# Autodesk Inventor assembly: папус для вари
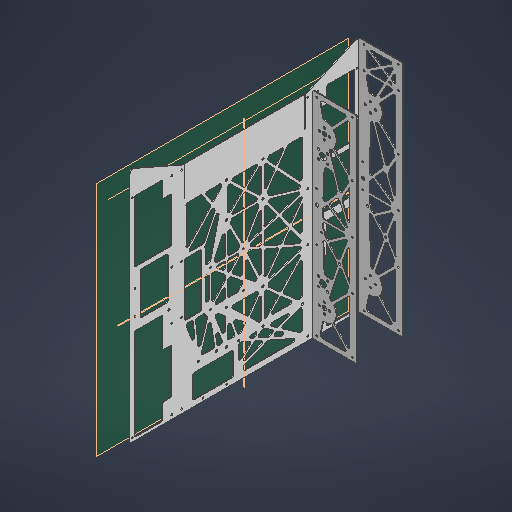
[picture p0: Inventor's stored thumbnail of the model, 512x512]
Saved by Autodesk Inventor 2026.2 (Build 302298000, 298)
## iProperties
Created: 2025-11-01
Part Number: папус для вари
Document SubType Name: Assembly
Designer: Phantom
Author: Phantom
## Documents named in this file (32)
- C:\Users\Phantom\Desktop\Phantom16950\папус для вари.iam
- C:\Users\Phantom\Desktop\Phantom16950\дно 25-26.ipt
- C:\Users\Phantom\Desktop\Phantom16950\кб 2025-2026.ipt
- C:\Users\Phantom\Desktop\Phantom16950\угол 25-26.ipt
- C:\Users\Phantom\Desktop\Phantom16950\кб 2025-2026 2 часть.ipt
- C:\Users\Phantom\Desktop\Phantom16950\кб 2025-2026 2 часть_MIR.ipt
- C:\Users\Phantom\Desktop\Phantom16950\ВЕРХ 25-26.ipt
- C:\Users\Phantom\Desktop\Phantom16950\наклон.ipt
- C:\Users\Phantom\Desktop\Phantom16950\цепь_MIR4.iam
- C:\Users\Phantom\Desktop\Phantom16950\КОЛЕСО_MIR_MIR3.ipt
- C:\Users\Phantom\Desktop\Phantom16950\арина треугольник 2.ipt
- C:\Users\Phantom\Desktop\Phantom16950\5203-2402-0014 assembly\5203-2402-0014 assembly.iam
- C:\Users\Phantom\Desktop\Phantom16950\шестерня шеврон кб 25-26.ipt
- C:\Users\Phantom\Desktop\Phantom16950\шестерня ответная 2.0 кб 25-26\шестерня ответная 2.0 кб 25-26.ipt
- C:\Users\Phantom\Desktop\Phantom16950\цепь_MIR4_MIR.iam
- C:\Users\Phantom\Desktop\Phantom16950\КОЛЕСО_MIR_MIR3_MIR.ipt
- C:\Users\Phantom\Desktop\Phantom16950\шестерня шеврон кб 25-26_MIR.ipt
- C:\Users\Phantom\Desktop\Phantom16950\шестерня ответная 2.0 кб 25-26\шестерня ответная 2.0 кб 25-26_MIR.ipt
- C:\Users\Phantom\Desktop\Phantom16950\цепь_MIR4_MIR1.iam
- C:\Users\Phantom\Desktop\Phantom16950\КОЛЕСО_MIR_MIR3_MIR1.ipt
- C:\Users\Phantom\Desktop\Phantom16950\шестерня шеврон кб 25-26_MIR1.ipt
- C:\Users\Phantom\Desktop\Phantom16950\шестерня ответная 2.0 кб 25-26\шестерня ответная 2.0 кб 25-26_MIR1.ipt
- C:\Users\Phantom\Desktop\Phantom16950\цепь_MIR4_MIR_MIR.iam
- C:\Users\Phantom\Desktop\Phantom16950\КОЛЕСО_MIR_MIR3_MIR_MIR.ipt
- C:\Users\Phantom\Desktop\Phantom16950\шестерня шеврон кб 25-26_MIR_MIR.ipt
- C:\Users\Phantom\Desktop\Phantom16950\шестерня ответная 2.0 кб 25-26\шестерня ответная 2.0 кб 25-26_MIR_MIR.ipt
- C:\Users\Phantom\Desktop\Phantom16950\вал кб.ipt
- C:\Users\Phantom\Desktop\Phantom16950\44260_txm_torquenado_dc_motor.ipt
- C:\Users\Phantom\Desktop\Phantom16950\подьем 25-26.iam
- C:\Users\Phantom\Desktop\Phantom16950\мотор подьем крепл 2 25-26.ipt
- C:\Users\Phantom\Desktop\Phantom16950\доп крепл мотора 25-26.ipt
- C:\Users\Phantom\Desktop\Phantom16950\крепл аккума 25-26 2 (2)\крепл аккума 25-26 2 (2)\крепл аккума 25-26 2 (2).ipt
## Components (53 placed, 31 different names)
1. дно 25-26:1 — Совмещение:15, Совмещение:17, Совмещение:20, Совмещение:22, Заподлицо:5, Заподлицо:8, Совмещение:97, Совмещение:99, Совмещение:101, Угол:1, Совмещение:104, Совмещение:106, Совмещение:107, Совмещение:109, Совмещение:110, Совмещение:112, Совмещение:114, Совмещение:116, Совмещение:118, Совмещение:120, Совмещение:122, Совмещение:126, Совмещение:127, Совмещение:129, Совмещение:131, Совмещение:133, Совмещение:136, Совмещение:137, Совмещение:138
2. кб 2025-2026:1 — Совмещение:14, Совмещение:16, Совмещение:21, Заподлицо:2, Заподлицо:3, Заподлицо:4, Заподлицо:6, Совмещение:48, Совмещение:60, Совмещение:73, Совмещение:88
3. угол 25-26:1 — Совмещение:16, Совмещение:17
4. угол 25-26:2 — Совмещение:14, Совмещение:15, Совмещение:20
5. кб 2025-2026 2 часть:1 — Совмещение:25, Совмещение:31, Совмещение:34, Совмещение:53, Совмещение:54, Совмещение:58, Совмещение:59, Совмещение:61, Совмещение:62, Совмещение:63, Совмещение:64, Совмещение:82, Совмещение:102, Совмещение:117, Совмещение:119, Совмещение:121, Совмещение:124, Совмещение:130, Совмещение:132
6. кб 2025-2026 2 часть_MIR:1 — Совмещение:25, Заподлицо:2, Заподлицо:3, Совмещение:27, Совмещение:31, Совмещение:38, Совмещение:39, Совмещение:60, Совмещение:65, Совмещение:66, Совмещение:71, Совмещение:72, Совмещение:96, Совмещение:108, Совмещение:123, Совмещение:125, Совмещение:128
7. кб 2025-2026:2 — Совмещение:21, Совмещение:24, Совмещение:59
8. угол 25-26:3 — Совмещение:22, Совмещение:24
9. угол 25-26:4 — Совмещение:27, Совмещение:107
10. угол 25-26:6 — Совмещение:34, Совмещение:122
11. ВЕРХ 25-26:1 — Совмещение:36, Заподлицо:4, Совмещение:55, Совмещение:88, Совмещение:105
12. угол 25-26:7 — Совмещение:38, Совмещение:39, Совмещение:36
13. наклон:1 — Совмещение:102, Совмещение:105, Совмещение:106
14. цепь_MIR4:1 [sub-assembly] — Совмещение:46, Совмещение:47, Совмещение:56, Совмещение:57, Совмещение:58
15. КОЛЕСО_MIR_MIR3:1 — Совмещение:46, Совмещение:47
16. арина треугольник 2:1 — Совмещение:48, Совмещение:104
17. 5203-2402-0014 assembly:1 [sub-assembly] — Совмещение:53, Совмещение:54, Совмещение:83
18. 5203-2402-0014 assembly:2 [sub-assembly] — Совмещение:135
19. шестерня шеврон кб 25-26:1 — Совмещение:56, Совмещение:57, Совмещение:61, Заподлицо:11, Заподлицо:15
20. шестерня ответная 2.0 кб 25-26:1 — Совмещение:62, Заподлицо:9, Заподлицо:12
21. 5203-2402-0014 assembly:3 [sub-assembly] — Совмещение:63, Совмещение:64, Совмещение:98
22. 5203-2402-0014 assembly:4 [sub-assembly] — Совмещение:65, Совмещение:66, Совмещение:100
23. цепь_MIR4_MIR:1 [sub-assembly] — Совмещение:67, Совмещение:68, Совмещение:69, Совмещение:70, Совмещение:71, Совмещение:73
24. КОЛЕСО_MIR_MIR3_MIR:1 — Совмещение:67, Совмещение:68
25. шестерня шеврон кб 25-26_MIR:1 — Совмещение:69, Совмещение:70, Заподлицо:12
26. шестерня ответная 2.0 кб 25-26_MIR:1 — Совмещение:72, Заподлицо:11
27. цепь_MIR4_MIR1:1 [sub-assembly] — Совмещение:74, Совмещение:75, Совмещение:76, Совмещение:77, Совмещение:82
28. КОЛЕСО_MIR_MIR3_MIR1:1 — Совмещение:74, Совмещение:75
29. шестерня шеврон кб 25-26_MIR1:1 — Совмещение:76, Совмещение:77, Заподлицо:14, Заподлицо:15
30. шестерня ответная 2.0 кб 25-26_MIR1:1 — Совмещение:83, Заподлицо:9, Заподлицо:13
31. цепь_MIR4_MIR_MIR:1 [sub-assembly] — Совмещение:78, Совмещение:79, Совмещение:80, Совмещение:81, Совмещение:123
32. КОЛЕСО_MIR_MIR3_MIR_MIR:1 — Совмещение:78, Совмещение:79
33. шестерня шеврон кб 25-26_MIR_MIR:1 — Совмещение:80, Совмещение:81, Заподлицо:13
34. шестерня ответная 2.0 кб 25-26_MIR_MIR:1 — Совмещение:124, Заподлицо:14
35. угол 25-26:8 — Совмещение:127, Совмещение:128
36. вал кб:1 — Совмещение:96
37. 44260_txm_torquenado_dc_motor:1 — Совмещение:113
38. подьем 25-26:1 [sub-assembly]
39. мотор подьем крепл 2 25-26:1 — Совмещение:97, Совмещение:114
40. доп крепл мотора 25-26:1 — Совмещение:98, Совмещение:99
41. доп крепл мотора 25-26:2 — Совмещение:100, Совмещение:101
42. угол 25-26:9 — Совмещение:108, Совмещение:109
43. мотор подьем крепл 2 25-26:2 — Совмещение:110, Совмещение:112, Совмещение:113
44. угол 25-26:10 — Совмещение:120, Совмещение:121
45. угол 25-26:11 — Совмещение:116, Совмещение:117
46. угол 25-26:12 — Совмещение:118, Совмещение:119, Совмещение:134
47. угол 25-26:13 — Совмещение:125, Совмещение:126
48. угол 25-26:14 — Совмещение:131, Совмещение:132
49. угол 25-26:15 — Совмещение:129, Совмещение:130
50. угол 25-26:16 — Совмещение:133, Совмещение:134
51. доп крепл мотора 25-26:3
52. доп крепл мотора 25-26:4 — Совмещение:135, Совмещение:136
53. крепл аккума 25-26 2 (2):1 — Совмещение:137, Совмещение:138
## Relationships (110: Mate 96, Flush 13, Angle 1)
- Совмещение:14 [Mate]: кб 2025-2026:1 ↔ угол 25-26:2
- Совмещение:15 [Mate]: дно 25-26:1 ↔ угол 25-26:2
- Совмещение:16 [Mate]: кб 2025-2026:1 ↔ угол 25-26:1
- Совмещение:17 [Mate]: дно 25-26:1 ↔ угол 25-26:1
- Совмещение:20 [Mate]: дно 25-26:1 ↔ угол 25-26:2
- Совмещение:21 [Mate]: кб 2025-2026:1 ↔ кб 2025-2026:2
- Совмещение:22 [Mate]: дно 25-26:1 ↔ угол 25-26:3
- Совмещение:24 [Mate]: кб 2025-2026:2 ↔ угол 25-26:3
- Совмещение:25 [Mate]: кб 2025-2026 2 часть:1 ↔ кб 2025-2026 2 часть_MIR:1
- Заподлицо:2 [Flush]: кб 2025-2026:1 ↔ кб 2025-2026 2 часть_MIR:1
- Заподлицо:3 [Flush]: кб 2025-2026:1 ↔ кб 2025-2026 2 часть_MIR:1
- Совмещение:27 [Mate]: кб 2025-2026 2 часть_MIR:1 ↔ угол 25-26:4
- Совмещение:31 [Mate]: кб 2025-2026 2 часть:1 ↔ кб 2025-2026 2 часть_MIR:1
- Совмещение:34 [Mate]: кб 2025-2026 2 часть:1 ↔ угол 25-26:6
- Совмещение:36 [Mate]: ВЕРХ 25-26:1 ↔ угол 25-26:7
- Заподлицо:4 [Flush]: кб 2025-2026:1 ↔ ВЕРХ 25-26:1
- Совмещение:38 [Mate]: кб 2025-2026 2 часть_MIR:1 ↔ угол 25-26:7
- Совмещение:39 [Mate] (2 mm): кб 2025-2026 2 часть_MIR:1 ↔ угол 25-26:7
- Заподлицо:5 [Flush] (25.725 mm): дно 25-26:1
- Заподлицо:6 [Flush] (-202.5 mm): кб 2025-2026:1
- Совмещение:46 [Mate]: цепь_MIR4:1 ↔ КОЛЕСО_MIR_MIR3:1
- Совмещение:47 [Mate]: цепь_MIR4:1 ↔ КОЛЕСО_MIR_MIR3:1
- Совмещение:48 [Mate]: кб 2025-2026:1 ↔ арина треугольник 2:1
- [Mate]: 5203-2402-0014 assembly:1 ↔ 5203-2402-0014 assembly:2
- [Flush]: 5203-2402-0014 assembly:1 ↔ 5203-2402-0014 assembly:2
- Совмещение:53 [Mate]: кб 2025-2026 2 часть:1 ↔ 5203-2402-0014 assembly:1
- Совмещение:54 [Mate]: кб 2025-2026 2 часть:1 ↔ 5203-2402-0014 assembly:1
- Совмещение:55 [Mate] (-195 mm): ВЕРХ 25-26:1
- Совмещение:56 [Mate]: цепь_MIR4:1 ↔ шестерня шеврон кб 25-26:1
- Совмещение:57 [Mate]: цепь_MIR4:1 ↔ шестерня шеврон кб 25-26:1
- Совмещение:58 [Mate]: кб 2025-2026 2 часть:1 ↔ цепь_MIR4:1
- Совмещение:59 [Mate] (80 mm): кб 2025-2026 2 часть:1 ↔ кб 2025-2026:2
- Совмещение:60 [Mate] (80 mm): кб 2025-2026:1 ↔ кб 2025-2026 2 часть_MIR:1
- Совмещение:61 [Mate] (9 mm): кб 2025-2026 2 часть:1 ↔ шестерня шеврон кб 25-26:1
- Совмещение:62 [Mate]: кб 2025-2026 2 часть:1 ↔ шестерня ответная 2.0 кб 25-26:1
- Совмещение:63 [Mate]: кб 2025-2026 2 часть:1 ↔ 5203-2402-0014 assembly:3
- Совмещение:64 [Mate]: кб 2025-2026 2 часть:1 ↔ 5203-2402-0014 assembly:3
- Совмещение:65 [Mate]: кб 2025-2026 2 часть_MIR:1 ↔ 5203-2402-0014 assembly:4
- Совмещение:66 [Mate]: кб 2025-2026 2 часть_MIR:1 ↔ 5203-2402-0014 assembly:4
- Совмещение:67 [Mate]: цепь_MIR4_MIR:1 ↔ КОЛЕСО_MIR_MIR3_MIR:1
- Совмещение:68 [Mate]: цепь_MIR4_MIR:1 ↔ КОЛЕСО_MIR_MIR3_MIR:1
- Совмещение:69 [Mate]: цепь_MIR4_MIR:1 ↔ шестерня шеврон кб 25-26_MIR:1
- Совмещение:70 [Mate]: цепь_MIR4_MIR:1 ↔ шестерня шеврон кб 25-26_MIR:1
- Совмещение:71 [Mate]: кб 2025-2026 2 часть_MIR:1 ↔ цепь_MIR4_MIR:1
- Совмещение:72 [Mate]: кб 2025-2026 2 часть_MIR:1 ↔ шестерня ответная 2.0 кб 25-26_MIR:1
- Совмещение:73 [Mate] (9 mm): кб 2025-2026:1 ↔ цепь_MIR4_MIR:1
- Заподлицо:8 [Flush] (-190 mm): дно 25-26:1
- Совмещение:74 [Mate]: цепь_MIR4_MIR1:1 ↔ КОЛЕСО_MIR_MIR3_MIR1:1
- Совмещение:75 [Mate]: цепь_MIR4_MIR1:1 ↔ КОЛЕСО_MIR_MIR3_MIR1:1
- Совмещение:76 [Mate]: цепь_MIR4_MIR1:1 ↔ шестерня шеврон кб 25-26_MIR1:1
- Совмещение:77 [Mate]: цепь_MIR4_MIR1:1 ↔ шестерня шеврон кб 25-26_MIR1:1
- Совмещение:78 [Mate]: цепь_MIR4_MIR_MIR:1 ↔ КОЛЕСО_MIR_MIR3_MIR_MIR:1
- Совмещение:79 [Mate]: цепь_MIR4_MIR_MIR:1 ↔ КОЛЕСО_MIR_MIR3_MIR_MIR:1
- Совмещение:80 [Mate]: цепь_MIR4_MIR_MIR:1 ↔ шестерня шеврон кб 25-26_MIR_MIR:1
- Совмещение:81 [Mate]: цепь_MIR4_MIR_MIR:1 ↔ шестерня шеврон кб 25-26_MIR_MIR:1
- Совмещение:82 [Mate]: кб 2025-2026 2 часть:1 ↔ цепь_MIR4_MIR1:1
- Совмещение:83 [Mate]: 5203-2402-0014 assembly:1 ↔ шестерня ответная 2.0 кб 25-26_MIR1:1
- Заподлицо:9 [Flush]: шестерня ответная 2.0 кб 25-26:1 ↔ шестерня ответная 2.0 кб 25-26_MIR1:1
- Совмещение:88 [Mate]: кб 2025-2026:1 ↔ ВЕРХ 25-26:1
- [Mate] (8 mm): 44260_txm_torquenado_dc_motor:1 ↔ подьем 25-26:1
- [Mate]: 44260_txm_torquenado_dc_motor:1 ↔ подьем 25-26:1
- [Mate]: 44260_txm_torquenado_dc_motor:1 ↔ мотор подьем крепл 2 25-26:1
- [Mate] (5 mm): 44260_txm_torquenado_dc_motor:1 ↔ мотор подьем крепл 2 25-26:1
- [Mate]: вал кб:1 ↔ подьем 25-26:1
- Совмещение:96 [Mate]: кб 2025-2026 2 часть_MIR:1 ↔ вал кб:1
- Совмещение:97 [Mate]: дно 25-26:1 ↔ мотор подьем крепл 2 25-26:1
- Совмещение:98 [Mate]: 5203-2402-0014 assembly:3 ↔ доп крепл мотора 25-26:1
- Совмещение:99 [Mate]: дно 25-26:1 ↔ доп крепл мотора 25-26:1
- Совмещение:100 [Mate]: 5203-2402-0014 assembly:4 ↔ доп крепл мотора 25-26:2
- Совмещение:101 [Mate]: дно 25-26:1 ↔ доп крепл мотора 25-26:2
- Совмещение:102 [Mate]: кб 2025-2026 2 часть:1 ↔ наклон:1
- Угол:1 [Angle] (0 deg): дно 25-26:1
- Совмещение:104 [Mate]: дно 25-26:1 ↔ арина треугольник 2:1
- Совмещение:105 [Mate]: ВЕРХ 25-26:1 ↔ наклон:1
- Совмещение:106 [Mate]: дно 25-26:1 ↔ наклон:1
- Совмещение:107 [Mate]: дно 25-26:1 ↔ угол 25-26:4
- Совмещение:108 [Mate]: кб 2025-2026 2 часть_MIR:1 ↔ угол 25-26:9
- Совмещение:109 [Mate]: дно 25-26:1 ↔ угол 25-26:9
- Совмещение:110 [Mate]: дно 25-26:1 ↔ мотор подьем крепл 2 25-26:2
- Совмещение:112 [Mate]: дно 25-26:1 ↔ мотор подьем крепл 2 25-26:2
- Совмещение:113 [Mate]: 44260_txm_torquenado_dc_motor:1 ↔ мотор подьем крепл 2 25-26:2
- Совмещение:114 [Mate]: дно 25-26:1 ↔ мотор подьем крепл 2 25-26:1
- Совмещение:116 [Mate]: дно 25-26:1 ↔ угол 25-26:11
- Совмещение:117 [Mate]: кб 2025-2026 2 часть:1 ↔ угол 25-26:11
- Совмещение:118 [Mate]: дно 25-26:1 ↔ угол 25-26:12
- Совмещение:119 [Mate]: кб 2025-2026 2 часть:1 ↔ угол 25-26:12
- Совмещение:120 [Mate]: дно 25-26:1 ↔ угол 25-26:10
- Совмещение:121 [Mate]: кб 2025-2026 2 часть:1 ↔ угол 25-26:10
- Совмещение:122 [Mate]: дно 25-26:1 ↔ угол 25-26:6
- Заподлицо:11 [Flush]: шестерня шеврон кб 25-26:1 ↔ шестерня ответная 2.0 кб 25-26_MIR:1
- Заподлицо:12 [Flush]: шестерня ответная 2.0 кб 25-26:1 ↔ шестерня шеврон кб 25-26_MIR:1
- Совмещение:123 [Mate]: кб 2025-2026 2 часть_MIR:1 ↔ цепь_MIR4_MIR_MIR:1
- Заподлицо:13 [Flush]: шестерня ответная 2.0 кб 25-26_MIR1:1 ↔ шестерня шеврон кб 25-26_MIR_MIR:1
- Совмещение:124 [Mate]: кб 2025-2026 2 часть:1 ↔ шестерня ответная 2.0 кб 25-26_MIR_MIR:1
- Заподлицо:14 [Flush]: шестерня шеврон кб 25-26_MIR1:1 ↔ шестерня ответная 2.0 кб 25-26_MIR_MIR:1
- Заподлицо:15 [Flush]: шестерня шеврон кб 25-26:1 ↔ шестерня шеврон кб 25-26_MIR1:1
- Совмещение:125 [Mate]: кб 2025-2026 2 часть_MIR:1 ↔ угол 25-26:13
- Совмещение:126 [Mate]: дно 25-26:1 ↔ угол 25-26:13
- Совмещение:127 [Mate]: дно 25-26:1 ↔ угол 25-26:8
- Совмещение:128 [Mate]: кб 2025-2026 2 часть_MIR:1 ↔ угол 25-26:8
- Совмещение:129 [Mate]: дно 25-26:1 ↔ угол 25-26:15
- Совмещение:130 [Mate]: кб 2025-2026 2 часть:1 ↔ угол 25-26:15
- Совмещение:131 [Mate]: дно 25-26:1 ↔ угол 25-26:14
- Совмещение:132 [Mate]: кб 2025-2026 2 часть:1 ↔ угол 25-26:14
- Совмещение:133 [Mate]: дно 25-26:1 ↔ угол 25-26:16
- Совмещение:134 [Mate]: угол 25-26:12 ↔ угол 25-26:16
- Совмещение:135 [Mate]: 5203-2402-0014 assembly:2 ↔ доп крепл мотора 25-26:4
- Совмещение:136 [Mate]: дно 25-26:1 ↔ доп крепл мотора 25-26:4
- Совмещение:137 [Mate]: дно 25-26:1 ↔ крепл аккума 25-26 2 (2):1
- Совмещение:138 [Mate]: дно 25-26:1 ↔ крепл аккума 25-26 2 (2):1
